# Autodesk Inventor assembly: akkum
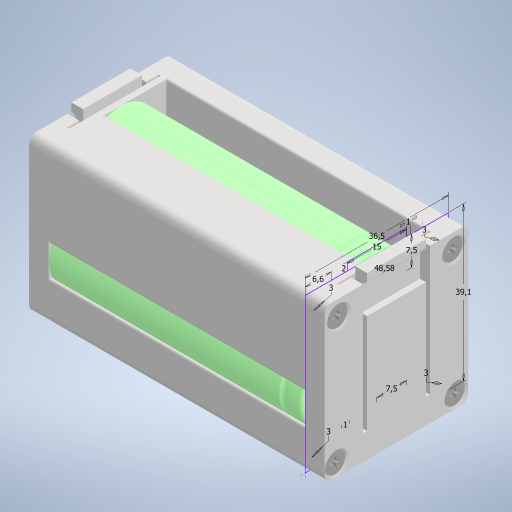
[picture p0: Inventor's stored thumbnail of the model, 512x512]
Saved by Autodesk Inventor 2023 (Build 270158000, 158)
## iProperties
Created: 2026-02-15
Part Number: akkum
Document SubType Name: Assembly
Designer: garin
Author: garin
## Documents named in this file (5)
- C:\Users\garin\OneDrive\Документы\maze\version1\akkum.iam
- C:\Users\garin\OneDrive\Документы\maze\version1\left_akkum.ipt
- C:\Users\garin\OneDrive\Документы\maze\version1\Generic Li Ion 1850 cell.ipt
- C:\Users\garin\OneDrive\Документы\maze\version1\akkum_wall.ipt
- C:\Users\garin\OneDrive\Документы\maze\version1\Винты M3 4 - 30 мм DIN965A 3D-модель.ipt
## Components (14 placed, 4 different names)
1. left_akkum:1 — Жесткий:1, Жесткий:2, Жесткий:3, Заподлицо:1, С поворотом:1
2. Generic Li Ion 1850 cell:1 — Жесткий:1
3. Generic Li Ion 1850 cell:2 — Жесткий:2
4. Generic Li Ion 1850 cell:3 — Жесткий:3
5. akkum_wall:1 — Заподлицо:1, С поворотом:2, С поворотом:3, Жесткий:4, С поворотом:4
6. akkum_wall:2 — С поворотом:1, С поворотом:5, Жесткий:5, С поворотом:6, С поворотом:7
7. Винты M3 4 - 30 мм DIN965A 3D-модель:1 — С поворотом:2
8. Винты M3 4 - 30 мм DIN965A 3D-модель:2 — С поворотом:3
9. Винты M3 4 - 30 мм DIN965A 3D-модель:3 — С поворотом:4
10. Винты M3 4 - 30 мм DIN965A 3D-модель:4 — Жесткий:4
11. Винты M3 4 - 30 мм DIN965A 3D-модель:5 — С поворотом:7
12. Винты M3 4 - 30 мм DIN965A 3D-модель:6 — С поворотом:6
13. Винты M3 4 - 30 мм DIN965A 3D-модель:7 — Жесткий:5
14. Винты M3 4 - 30 мм DIN965A 3D-модель:8 — С поворотом:5
## Relationships (13: RevoluteJoint 7, WeldJoint 5, Flush 1)
- Жесткий:1 [WeldJoint]: left_akkum:1 ↔ Generic Li Ion 1850 cell:1
- Жесткий:2 [WeldJoint]: left_akkum:1 ↔ Generic Li Ion 1850 cell:2
- Жесткий:3 [WeldJoint]: left_akkum:1 ↔ Generic Li Ion 1850 cell:3
- Заподлицо:1 [Flush]: left_akkum:1 ↔ akkum_wall:1
- С поворотом:1 [RevoluteJoint]: left_akkum:1 ↔ akkum_wall:2
- С поворотом:2 [RevoluteJoint]: akkum_wall:1 ↔ Винты M3 4 - 30 мм DIN965A 3D-модель:1
- С поворотом:3 [RevoluteJoint]: akkum_wall:1 ↔ Винты M3 4 - 30 мм DIN965A 3D-модель:2
- Жесткий:4 [WeldJoint]: akkum_wall:1 ↔ Винты M3 4 - 30 мм DIN965A 3D-модель:4
- С поворотом:4 [RevoluteJoint]: akkum_wall:1 ↔ Винты M3 4 - 30 мм DIN965A 3D-модель:3
- С поворотом:5 [RevoluteJoint]: akkum_wall:2 ↔ Винты M3 4 - 30 мм DIN965A 3D-модель:8
- Жесткий:5 [WeldJoint]: akkum_wall:2 ↔ Винты M3 4 - 30 мм DIN965A 3D-модель:7
- С поворотом:6 [RevoluteJoint]: akkum_wall:2 ↔ Винты M3 4 - 30 мм DIN965A 3D-модель:6
- С поворотом:7 [RevoluteJoint]: akkum_wall:2 ↔ Винты M3 4 - 30 мм DIN965A 3D-модель:5
